# Autodesk Inventor assembly: COTS_GENERIC_80x80x25_Fan
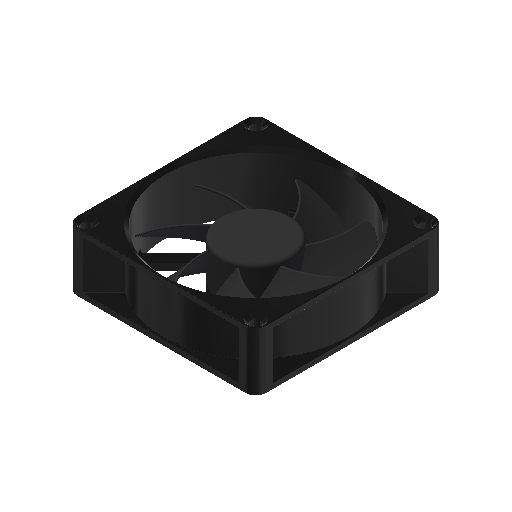
[picture p0: Inventor's stored thumbnail of the model, 512x512]
Saved by Autodesk Inventor 2026.1 (Build 301233000, 233)
## iProperties
Created: 2015-03-08
Part Number: COTS_GENERIC_80x80x25_Fan
Document SubType Name: Assembly
Designer: Venci
Author: Venci
## Documents named in this file (3)
- C:\Users\Andrzej\OneDrive\_DRIVE_SYNCH_FILES\__ BYTECHLAB PROJECTS\MECH - FDM 3D Printer - RAPTOR-360\MCAD\1_REV1\__COTS_PARTS\COTS_GENERIC_80x80x25_Fan\COTS_GENERIC_80x80x25_Fan.iam
- C:\Users\Andrzej\OneDrive\_DRIVE_SYNCH_FILES\__ BYTECHLAB PROJECTS\MECH - FDM 3D Printer - RAPTOR-360\MCAD\1_REV1\__COTS_PARTS\COTS_GENERIC_80x80x25_Fan\sunon_frame.ipt
- C:\Users\Andrzej\OneDrive\_DRIVE_SYNCH_FILES\__ BYTECHLAB PROJECTS\MECH - FDM 3D Printer - RAPTOR-360\MCAD\1_REV1\__COTS_PARTS\COTS_GENERIC_80x80x25_Fan\sunon_blade_80.ipt
## Components (2 placed, 2 different names)
1. sunon_frame:1 — Insert:1
2. sunon_blade_80:1 — Insert:1
## Relationships (1: Insert 1)
- Insert:1: sunon_frame:1 ↔ sunon_blade_80:1
